# Autodesk Inventor assembly: turn encoder assembly 2
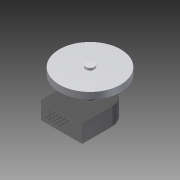
[picture p0: Inventor's stored thumbnail of the model, 180x180]
Saved by Autodesk Inventor 2012 (Build 160160000, 160)
## iProperties
Created: 2012-07-13
Part Number: turn encoder assembly 2
Document SubType Name: Assembly
Designer: Bryce
Author: Bryce
## Documents named in this file (3)
- C:\Users\Bryce\Dropbox\Inventor Design Project Files\Independent Swerves\Inventor 2012\turn encoder assembly 2.iam
- C:\Users\Bryce\Dropbox\Inventor Design Project Files\Independent Swerves\Imported Components\Encoder USD S1-100-B Assy.iam
- C:\Users\Bryce\Dropbox\Inventor Design Project Files\Independent Swerves\Imported Components\a_1m_2-y24054\a_1m_2-y24054 2.ipt
## Components (2 placed, 2 different names)
1. Encoder USD S1-100-B Assy:1 [sub-assembly] — Mate:5, Mate:6
2. a_1m_2-y24054 2:1 — Mate:5, Mate:6
## Relationships (2: Mate 2)
- Mate:5: Encoder USD S1-100-B Assy:1 ↔ a_1m_2-y24054 2:1
- Mate:6: Encoder USD S1-100-B Assy:1 ↔ a_1m_2-y24054 2:1
